# Autodesk Inventor assembly: MAIN Gripper assembly
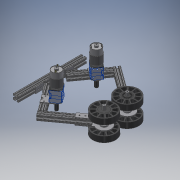
[picture p0: Inventor's stored thumbnail of the model, 180x180]
Saved by Autodesk Inventor 2018 (Build 220112000, 112)
## iProperties
Created: 2019-01-25
Part Number: MAIN Gripper assembly
Document SubType Name: Assembly
Designer: s-2513225
Author: s-2513225
## Documents named in this file (4)
- E:\Robotics\Ball Intake ver 2\MAIN Gripper assembly.iam
- E:\Robotics\Ball Intake ver 2\left arm.iam
- E:\Robotics\Ball Intake ver 2\right arm.iam
- E:\Robotics\Ball Intake ver 2\1010.IPT
## Components (3 placed, 3 different names)
1. left arm:1 [sub-assembly] — Mate:1, Flush:2
2. right arm:1 [sub-assembly] — Mate:2, Flush:1
3. 1010:1 — Mate:1, Mate:2, Flush:1, Flush:2
## Relationships (4: Mate 2, Flush 2)
- Mate:1: left arm:1 ↔ 1010:1
- Mate:2: right arm:1 ↔ 1010:1
- Flush:1: right arm:1 ↔ 1010:1
- Flush:2: left arm:1 ↔ 1010:1
